# Autodesk Inventor assembly: Ensamblaje1
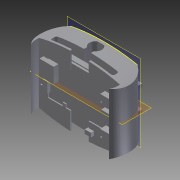
[picture p0: Inventor's stored thumbnail of the model, 180x180]
Saved by Autodesk Inventor 2012 (Build 160160000, 160)
## iProperties
Created: 2012-12-28
Part Number: Ensamblaje1
Document SubType Name: Assembly
Designer: otrebor
Author: otrebor
## Documents named in this file (5)
- C:\Users\asimov\Documents\GitHub\modi\Hardware\Inventor 2012\Ensamblaje1.iam
- C:\Users\asimov\Documents\GitHub\modi\Hardware\Inventor 2012\chasis.ipt
- C:\Users\asimov\Documents\GitHub\modi\Hardware\Inventor 2012\bateria.ipt
- C:\Users\asimov\Documents\GitHub\modi\Hardware\Inventor 2012\fio.ipt
- C:\Users\asimov\Documents\GitHub\modi\Hardware\Inventor 2012\lipoRiderPro.ipt
## Components (4 placed, 4 different names)
1. chasis:1 — Coincidencia:1, Flush:1
2. bateria:1 — Coincidencia:3
3. fio:1 — Coincidencia:1, Flush:1
4. lipoRiderPro:1 — Coincidencia:3
## Relationships (3: Mate 2, Flush 1)
- Coincidencia:1 [Mate]: chasis:1 ↔ fio:1
- Coincidencia:3 [Mate]: bateria:1 ↔ lipoRiderPro:1
- Flush:1: chasis:1 ↔ fio:1
